# Autodesk Inventor assembly: MS_R_FrontLayer_v3
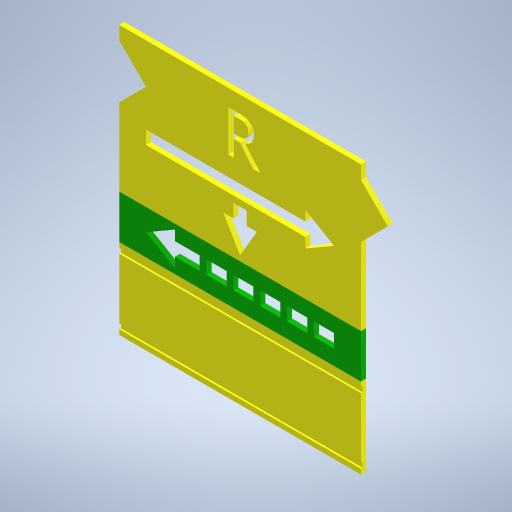
[picture p0: Inventor's stored thumbnail of the model, 512x512]
Saved by Autodesk Inventor 2024 (Build 280153000, 153)
## iProperties
Created: 2024-04-12
Part Number: MS_R_FrontLayer_v3
Document SubType Name: Assembly
Designer: LKLM
Author: LKLM
## Documents named in this file (4)
- C:\Data\Gitlab\ucl-aef-rdlab\RIG\V3\R\MS_R_FrontLayer_v3.iam
- C:\Data\Gitlab\ucl-aef-rdlab\RIG\V3\R\MS_R_FrontLayer_Yellow_Top_v3.ipt
- C:\Data\Gitlab\ucl-aef-rdlab\RIG\V3\R\MS_R_FrontLayer_Yellow_Green_Middle_v3.ipt
- C:\Data\Gitlab\ucl-aef-rdlab\RIG\V3\R\MS_R_FrontLayer_Yellow_Bottom_v3.ipt
## Components (3 placed, 3 different names)
1. MS_R_FrontLayer_Yellow_Top_v3:1 — Rigid:1
2. MS_R_FrontLayer_Yellow_Green_Middle_v3:1 — Rigid:1, Rigid:2
3. MS_R_FrontLayer_Yellow_Bottom_v3:1 — Rigid:2
## Relationships (2: WeldJoint 2)
- Rigid:1 [WeldJoint]: MS_R_FrontLayer_Yellow_Top_v3:1 ↔ MS_R_FrontLayer_Yellow_Green_Middle_v3:1
- Rigid:2 [WeldJoint]: MS_R_FrontLayer_Yellow_Green_Middle_v3:1 ↔ MS_R_FrontLayer_Yellow_Bottom_v3:1
